# Autodesk Inventor assembly: ControlBox
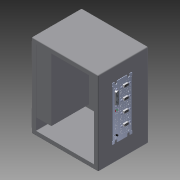
[picture p0: Inventor's stored thumbnail of the model, 180x180]
Saved by Autodesk Inventor 2013 (Build 170138000, 138)
## iProperties
Created: 2013-01-14
Part Number: ControlBox
Document SubType Name: Assembly
Designer: Istvan
Author: Istvan
## Documents named in this file (4)
- E:\GitHub\Crown-Fire\CAD\Electronics\ControlBox.iam
- E:\GitHub\Crown-Fire\CAD\Electronics\Enclosure\enclosure.iam
- E:\GitHub\Crown-Fire\CAD\Electronics\Controller\Geckdrive G540\Geckdrive G540.iam
- E:\GitHub\Crown-Fire\CAD\Electronics\powerSupply.ipt
## Components (3 placed, 3 different names)
1. enclosure:1 [sub-assembly] — Mate:1, Mate:2, Mate:3, Mate:4, Mate:5, Mate:6
2. Geckdrive G540:1 [sub-assembly] — Mate:1, Mate:2, Mate:3
3. powerSupply:1 — Mate:4, Mate:5, Mate:6
## Relationships (6: Mate 6)
- Mate:1: enclosure:1 ↔ Geckdrive G540:1
- Mate:2: enclosure:1 ↔ Geckdrive G540:1
- Mate:3: enclosure:1 ↔ Geckdrive G540:1
- Mate:4: enclosure:1 ↔ powerSupply:1
- Mate:5: enclosure:1 ↔ powerSupply:1
- Mate:6 (6.35 mm): enclosure:1 ↔ powerSupply:1
